# Autodesk Inventor assembly: ASY MSC 500 BELLY
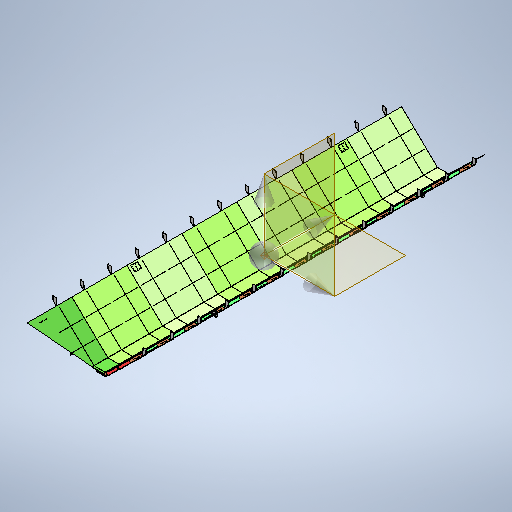
[picture p0: Inventor's stored thumbnail of the model, 512x512]
Saved by Autodesk Inventor 2025.1 (Build 291241020, 241B)
## iProperties
Created: 2024-07-22
Part Number: ASY MSC 500 BELLY
Document SubType Name: Assembly
Designer: pokla
Stock Number: ASY МОО 500 брюхо
Mass: 364753 g
Surface Area: 330564 cm^2
Volume: 45594.1 cm^3
Author: pokla
## Documents named in this file (8)
- C:\Users\user\YandexDisk-badmisterfox\домашниий пк\Inventor\Manturovo\Manturovo_Se-clar\ASY MSC 500 BELLY.iam
- C:\Users\user\YandexDisk-badmisterfox\домашниий пк\Inventor\Manturovo\Manturovo_Se-clar\MSC 501 sheet belly main.ipt
- C:\Users\user\YandexDisk-badmisterfox\домашниий пк\Inventor\Manturovo\Manturovo_Se-clar\MSC 502 sheet belly-neck.ipt
- C:\Users\user\YandexDisk-badmisterfox\домашниий пк\Inventor\Manturovo\Manturovo_Se-clar\MSC 504 stringer board belly.ipt
- C:\Users\user\YandexDisk-badmisterfox\домашниий пк\Inventor\Manturovo\Manturovo_Se-clar\MSC 503 rib belly.ipt
- C:\Users\user\YandexDisk-badmisterfox\домашниий пк\Inventor\Manturovo\Manturovo_Se-clar\MSC 505 STRINGER BOARD BELLY FACE.ipt
- C:\Users\user\YandexDisk-badmisterfox\домашниий пк\Inventor\Manturovo\Manturovo_Se-clar\MSC 506 STRINGER BOARD BELLY.ipt
- C:\Users\user\YandexDisk-badmisterfox\домашниий пк\Inventor\Manturovo\Manturovo_Se-clar\ASY MSC D-ring.iam
## Components (91 placed, 7 different names)
1. ASY MSC D-ring:1 [sub-assembly] — Mate:29, Mate:30
2. ASY MSC D-ring:2 [sub-assembly] — Mate:28, Mate:31
3. ASY MSC D-ring:3 [sub-assembly] — Mate:27, Mate:33
4. ASY MSC D-ring:4 [sub-assembly] — Mate:26, Mate:32
5. MSC 502 sheet belly-neck.ipt:1 — Rigid:24
6. MSC 501 sheet belly main.ipt:5 — Rigid:24, Mate:30, Mate:33
7. MSC 501 sheet belly main.ipt:4 — Mate:27, Mate:29
8. MSC 501 sheet belly main.ipt:3
9. MSC 501 sheet belly main.ipt:1
10. MSC 501 sheet belly main.ipt:2 — Mate:26, Mate:28, Mate:31
11. MSC 501 sheet belly main.ipt:6 — Mate:4, Mate:5, Mate:6, Mate:7, Flush:1, Mate:9, Mate:10, Flush:2, Mate:11, Mate:12, Mate:32
12. MSC 503 rib belly.ipt:1 — Rigid:17, Rigid:20, Rigid:21, Mate:13, Mate:17, Mate:20, Mate:21
13. MSC 503 rib belly.ipt:2 — Rigid:18, Rigid:19, Mate:11, Mate:12, Mate:13, Mate:14, Mate:18, Mate:19
14. MSC 504 stringer board belly.ipt:1 — Rigid:21, Flush:2
15. MSC 504 stringer board belly.ipt:2 — Rigid:20
16. MSC 504 stringer board belly.ipt:3 — Rigid:19
17. MSC 504 stringer board belly.ipt:4 — Rigid:18
18. MSC 505 STRINGER BOARD BELLY FACE.ipt:1 — Rigid:25
19. MSC 505 STRINGER BOARD BELLY FACE.ipt:2 — Rigid:26
20. MSC 505 STRINGER BOARD BELLY FACE.ipt:3
21. MSC 505 STRINGER BOARD BELLY FACE.ipt:4 — Rigid:28
22. MSC 506 STRINGER BOARD BELLY.ipt:25 — Mate:14, Mate:18, Mate:19, Rigid:29
23. MSC 506 STRINGER BOARD BELLY.ipt:26 — Mate:17, Rigid:30, Mate:20, Mate:21
24. MSC 504 stringer board belly.ipt:5
25. MSC 504 stringer board belly.ipt:6
26. MSC 504 stringer board belly.ipt:7
27. MSC 504 stringer board belly.ipt:8
28. MSC 504 stringer board belly.ipt:9
29. MSC 504 stringer board belly.ipt:10
30. MSC 504 stringer board belly.ipt:11
31. MSC 504 stringer board belly.ipt:12
32. MSC 504 stringer board belly.ipt:13
33. MSC 504 stringer board belly.ipt:14
34. MSC 504 stringer board belly.ipt:15
35. MSC 504 stringer board belly.ipt:16
36. MSC 504 stringer board belly.ipt:17
37. MSC 504 stringer board belly.ipt:18
38. MSC 504 stringer board belly.ipt:19
39. MSC 504 stringer board belly.ipt:20
40. MSC 504 stringer board belly.ipt:21 — Rigid:28
41. MSC 504 stringer board belly.ipt:22
42. MSC 504 stringer board belly.ipt:23 — Rigid:25
43. MSC 504 stringer board belly.ipt:24 — Rigid:26
44. MSC 503 rib belly.ipt:3 — Mate:6, Mate:7, Mate:8, Rigid:17
45. MSC 503 rib belly.ipt:4 — Mate:4, Mate:5, Mate:8
46. MSC 506 STRINGER BOARD BELLY.ipt:1 — Rigid:30
47. MSC 506 STRINGER BOARD BELLY.ipt:2 — Rigid:29
48. MSC 503 rib belly.ipt:5
49. MSC 503 rib belly.ipt:6
50. MSC 506 STRINGER BOARD BELLY.ipt:3
51. MSC 506 STRINGER BOARD BELLY.ipt:4
52. MSC 503 rib belly.ipt:7
53. MSC 503 rib belly.ipt:8
54. MSC 506 STRINGER BOARD BELLY.ipt:5
55. MSC 506 STRINGER BOARD BELLY.ipt:6
56. MSC 503 rib belly.ipt:9
57. MSC 503 rib belly.ipt:10
58. MSC 506 STRINGER BOARD BELLY.ipt:7
59. MSC 506 STRINGER BOARD BELLY.ipt:8
60. MSC 503 rib belly.ipt:11
61. MSC 503 rib belly.ipt:12
62. MSC 506 STRINGER BOARD BELLY.ipt:9
63. MSC 506 STRINGER BOARD BELLY.ipt:10
64. MSC 503 rib belly.ipt:13
65. MSC 503 rib belly.ipt:14
66. MSC 506 STRINGER BOARD BELLY.ipt:11
67. MSC 506 STRINGER BOARD BELLY.ipt:12
68. MSC 503 rib belly.ipt:15
69. MSC 503 rib belly.ipt:16
70. MSC 506 STRINGER BOARD BELLY.ipt:13
71. MSC 506 STRINGER BOARD BELLY.ipt:14
72. MSC 503 rib belly.ipt:17
73. MSC 503 rib belly.ipt:18
74. MSC 506 STRINGER BOARD BELLY.ipt:15
75. MSC 506 STRINGER BOARD BELLY.ipt:16
76. MSC 503 rib belly.ipt:19
77. MSC 503 rib belly.ipt:20
78. MSC 506 STRINGER BOARD BELLY.ipt:17
79. MSC 506 STRINGER BOARD BELLY.ipt:18
80. MSC 503 rib belly.ipt:21
81. MSC 503 rib belly.ipt:22
82. MSC 506 STRINGER BOARD BELLY.ipt:19
83. MSC 506 STRINGER BOARD BELLY.ipt:20
84. MSC 503 rib belly.ipt:23
85. MSC 503 rib belly.ipt:24
86. MSC 506 STRINGER BOARD BELLY.ipt:21
87. MSC 506 STRINGER BOARD BELLY.ipt:22
88. MSC 503 rib belly.ipt:25
89. MSC 503 rib belly.ipt:26
90. MSC 506 STRINGER BOARD BELLY.ipt:23
91. MSC 506 STRINGER BOARD BELLY.ipt:24
## Component patterns: (5 elements, first: MSC 504 stringer board belly.ipt:5 + MSC 504 stringer board belly.ipt:6 + MSC 504 stringer board belly.ipt:7 + MSC 504 stringer board belly.ipt:8), (12 elements, first: MSC 503 rib belly.ipt:3 + MSC 503 rib belly.ipt:4 + MSC 506 STRINGER BOARD BELLY.ipt:1 + MSC 506 STRINGER BOARD BELLY.ipt:2)
## Relationships (50: Mate 28, WeldJoint 20, Flush 2)
- [WeldJoint]: MSC 501 sheet belly main.ipt:1 ↔ MSC 501 sheet belly main.ipt:2
- [WeldJoint]: MSC 501 sheet belly main.ipt:3 ↔ MSC 501 sheet belly main.ipt:1
- [WeldJoint]: MSC 501 sheet belly main.ipt:5 ↔ MSC 501 sheet belly main.ipt:4
- [WeldJoint]: MSC 501 sheet belly main.ipt:4 ↔ MSC 501 sheet belly main.ipt:3
- [WeldJoint]: MSC 501 sheet belly main.ipt:2 ↔ MSC 501 sheet belly main.ipt:6
- [WeldJoint]: MSC 504 stringer board belly.ipt:3 ↔ MSC 504 stringer board belly.ipt:5
- [WeldJoint]: MSC 504 stringer board belly.ipt:4 ↔ MSC 504 stringer board belly.ipt:6
- [WeldJoint]: MSC 504 stringer board belly.ipt:2 ↔ MSC 504 stringer board belly.ipt:7
- [WeldJoint]: MSC 504 stringer board belly.ipt:1 ↔ MSC 504 stringer board belly.ipt:8
- Mate:4: MSC 501 sheet belly main.ipt:6 ↔ MSC 503 rib belly.ipt:4
- Mate:5: MSC 501 sheet belly main.ipt:6 ↔ MSC 503 rib belly.ipt:4
- Mate:6: MSC 501 sheet belly main.ipt:6 ↔ MSC 503 rib belly.ipt:3
- Mate:7: MSC 501 sheet belly main.ipt:6 ↔ MSC 503 rib belly.ipt:3
- Mate:8: MSC 503 rib belly.ipt:3 ↔ MSC 503 rib belly.ipt:4
- Flush:1: MSC 501 sheet belly main.ipt:6
- Mate:9: MSC 501 sheet belly main.ipt:6
- Mate:10: MSC 501 sheet belly main.ipt:6
- Rigid:17 [WeldJoint] (490 mm): MSC 503 rib belly.ipt:1 ↔ MSC 503 rib belly.ipt:3
- Rigid:18 [WeldJoint]: MSC 503 rib belly.ipt:2 ↔ MSC 504 stringer board belly.ipt:4
- Rigid:19 [WeldJoint]: MSC 503 rib belly.ipt:2 ↔ MSC 504 stringer board belly.ipt:3
- Rigid:20 [WeldJoint]: MSC 503 rib belly.ipt:1 ↔ MSC 504 stringer board belly.ipt:2
- Rigid:21 [WeldJoint]: MSC 503 rib belly.ipt:1 ↔ MSC 504 stringer board belly.ipt:1
- Flush:2: MSC 501 sheet belly main.ipt:6 ↔ MSC 504 stringer board belly.ipt:1
- Mate:11: MSC 501 sheet belly main.ipt:6 ↔ MSC 503 rib belly.ipt:2
- Mate:12: MSC 501 sheet belly main.ipt:6 ↔ MSC 503 rib belly.ipt:2
- Mate:13: MSC 503 rib belly.ipt:1 ↔ MSC 503 rib belly.ipt:2
- Rigid:24 [WeldJoint]: MSC 502 sheet belly-neck.ipt:1 ↔ MSC 501 sheet belly main.ipt:5
- Rigid:25 [WeldJoint]: MSC 505 STRINGER BOARD BELLY FACE.ipt:1 ↔ MSC 504 stringer board belly.ipt:23
- Rigid:26 [WeldJoint]: MSC 505 STRINGER BOARD BELLY FACE.ipt:2 ↔ MSC 504 stringer board belly.ipt:24
- Rigid:28 [WeldJoint]: MSC 505 STRINGER BOARD BELLY FACE.ipt:4 ↔ MSC 504 stringer board belly.ipt:21
- Mate:14: MSC 503 rib belly.ipt:2 ↔ MSC 506 STRINGER BOARD BELLY.ipt:25
- Mate:17 (-30 mm): MSC 503 rib belly.ipt:1 ↔ MSC 506 STRINGER BOARD BELLY.ipt:26
- Mate:18: MSC 503 rib belly.ipt:2 ↔ MSC 506 STRINGER BOARD BELLY.ipt:25
- Mate:19 (-20 mm): MSC 503 rib belly.ipt:2 ↔ MSC 506 STRINGER BOARD BELLY.ipt:25
- Rigid:29 [WeldJoint] (-490 mm): MSC 506 STRINGER BOARD BELLY.ipt:25 ↔ MSC 506 STRINGER BOARD BELLY.ipt:2
- Rigid:30 [WeldJoint] (-490 mm): MSC 506 STRINGER BOARD BELLY.ipt:26 ↔ MSC 506 STRINGER BOARD BELLY.ipt:1
- Mate:20: MSC 503 rib belly.ipt:1 ↔ MSC 506 STRINGER BOARD BELLY.ipt:26
- Mate:21: MSC 503 rib belly.ipt:1 ↔ MSC 506 STRINGER BOARD BELLY.ipt:26
- [Mate]: ASY MSC D-ring:1 ↔ MSC 501 sheet belly main.ipt:4
- [Mate]: ASY MSC D-ring:2 ↔ MSC 501 sheet belly main.ipt:2
- [Mate]: ASY MSC D-ring:4 ↔ MSC 501 sheet belly main.ipt:2
- [Mate]: ASY MSC D-ring:3 ↔ MSC 501 sheet belly main.ipt:4
- Mate:26 (-25 mm): ASY MSC D-ring:4 ↔ MSC 501 sheet belly main.ipt:2
- Mate:27 (-25 mm): ASY MSC D-ring:3 ↔ MSC 501 sheet belly main.ipt:4
- Mate:28 (-25 mm): ASY MSC D-ring:2 ↔ MSC 501 sheet belly main.ipt:2
- Mate:29 (-25 mm): ASY MSC D-ring:1 ↔ MSC 501 sheet belly main.ipt:4
- Mate:30 (50 mm): ASY MSC D-ring:1 ↔ MSC 501 sheet belly main.ipt:5
- Mate:31 (50 mm): ASY MSC D-ring:2 ↔ MSC 501 sheet belly main.ipt:2
- Mate:32 (50 mm): ASY MSC D-ring:4 ↔ MSC 501 sheet belly main.ipt:6
- Mate:33 (50 mm): ASY MSC D-ring:3 ↔ MSC 501 sheet belly main.ipt:5
